# Autodesk Inventor assembly: final assembly
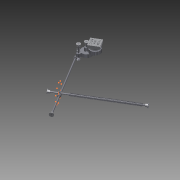
[picture p0: Inventor's stored thumbnail of the model, 180x180]
Saved by Autodesk Inventor 2011 (Build 150239000, 239)
## iProperties
Created: 2011-11-27
Part Number: final assembly
Document SubType Name: Assembly
Designer: Tom
Author: Tom
## Documents named in this file (8)
- E:\3\final assembly.iam
- E:\3\New CD RH Motor.ipt
- E:\3\Spur Gears3.iam
- E:\3\Worm Gears2.iam
- E:\3\Worm Gears5.iam
- E:\3\Spur Gears1.iam
- E:\3\Worm Gears3.iam
- E:\3\Part4.ipt
## Components (12 placed, 4 different names)
1. New CD RH Motor:1 — Angle:1, Angle:2, Mate:2, Flush:1, Rotation:2, Angle:3, Flush:9, Rotation:5
2. Spur Gears:1 [sub-assembly] — Mate:2, Flush:1, Flush:2, Rotation:2, Rotation:4, Mate:13, Flush:7, Flush:9, Rotation:5, Rotation:8
3. Worm Gears:1 [sub-assembly] — Angle:1, Angle:2, Mate:5, Rotation:3, Mate:9, Flush:3, Mate:14, Flush:8, Mate:15, Mate:16, Rotation:7, Mate:17, Rotation:10
4. Worm Gears:3 [sub-assembly] — Mate:8, Rotation:6, Mate:18, Rotation:11
5. Spur Gears:2 [sub-assembly] — Flush:2, Mate:5, Rotation:3, Rotation:4, Flush:6, Mate:12, Rotation:9, Mate:17
6. Worm Gears:5 [sub-assembly] — Angle:3, Mate:8, Mate:9, Mate:10, Flush:4, Mate:11, Flush:5, Mate:16, Mate:18, Rotation:11, Rotation:12
7. Part4:1 — Flush:3, Mate:15, Rotation:10
8. Part4:2 — Mate:10, Flush:4, Rotation:6
9. Part4:3 — Mate:11, Flush:5, Rotation:12
10. Part4:4 — Flush:6, Mate:12, Rotation:9
11. Part4:5 — Mate:13, Flush:7, Rotation:8
12. Part4:6 — Mate:14, Flush:8, Rotation:7
## Relationships (36: Mate 13, RelateRotation 11, Flush 9, Angle 3)
- Angle:1 (0 deg): New CD RH Motor:1 ↔ Worm Gears:1
- Angle:2 (90 deg): New CD RH Motor:1 ↔ Worm Gears:1
- Mate:2: New CD RH Motor:1 ↔ Spur Gears:1
- Flush:1: New CD RH Motor:1 ↔ Spur Gears:1
- Flush:2: Spur Gears:1 ↔ Spur Gears:2
- Mate:5: Worm Gears:1 ↔ Spur Gears:2
- Rotation:2 [RelateRotation] (1 ul): New CD RH Motor:1 ↔ Spur Gears:1
- Rotation:3 [RelateRotation] (1 ul): Worm Gears:1 ↔ Spur Gears:2
- Rotation:4 [RelateRotation] (1 ul): Spur Gears:1 ↔ Spur Gears:2
- Angle:3 (0 deg): New CD RH Motor:1 ↔ Worm Gears:5
- Mate:8 (10 mm): Worm Gears:3 ↔ Worm Gears:5
- Mate:9 (72 mm): Worm Gears:1 ↔ Worm Gears:5
- Flush:3: Worm Gears:1 ↔ Part4:1
- Mate:10: Worm Gears:5 ↔ Part4:2
- Flush:4: Worm Gears:5 ↔ Part4:2
- Mate:11: Worm Gears:5 ↔ Part4:3
- Flush:5: Worm Gears:5 ↔ Part4:3
- Flush:6: Spur Gears:2 ↔ Part4:4
- Mate:12: Spur Gears:2 ↔ Part4:4
- Mate:13: Spur Gears:1 ↔ Part4:5
- Flush:7: Spur Gears:1 ↔ Part4:5
- Mate:14: Worm Gears:1 ↔ Part4:6
- Flush:8: Worm Gears:1 ↔ Part4:6
- Mate:15: Worm Gears:1 ↔ Part4:1
- Mate:16: Worm Gears:1 ↔ Worm Gears:5
- Flush:9: New CD RH Motor:1 ↔ Spur Gears:1
- Rotation:5 [RelateRotation] (1 ul): New CD RH Motor:1 ↔ Spur Gears:1
- Rotation:6 [RelateRotation] (1 ul): Worm Gears:3 ↔ Part4:2
- Rotation:7 [RelateRotation] (1 ul): Worm Gears:1 ↔ Part4:6
- Rotation:8 [RelateRotation] (1 ul): Spur Gears:1 ↔ Part4:5
- Rotation:9 [RelateRotation] (2 ul): Spur Gears:2 ↔ Part4:4
- Mate:17: Worm Gears:1 ↔ Spur Gears:2
- Mate:18: Worm Gears:3 ↔ Worm Gears:5
- Rotation:10 [RelateRotation] (1 ul): Worm Gears:1 ↔ Part4:1
- Rotation:11 [RelateRotation] (1 ul): Worm Gears:3 ↔ Worm Gears:5
- Rotation:12 [RelateRotation] (1 ul): Worm Gears:5 ↔ Part4:3
